# Autodesk Inventor assembly: camMounted
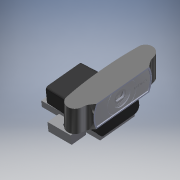
[picture p0: Inventor's stored thumbnail of the model, 180x180]
Saved by Autodesk Inventor 2017 (Build 210142000, 142)
## iProperties
Created: 2017-03-20
Part Number: camMounted
Document SubType Name: Assembly
Designer: Naga
Author: Naga
## Documents named in this file (3)
- E:\GDrive\IEEE CS\SoutheastCon2017\Cad\Electronics\camera\camMounted.iam
- E:\GDrive\IEEE CS\SoutheastCon2017\Cad\Electronics\camera\mount.ipt
- E:\GDrive\IEEE CS\SoutheastCon2017\Cad\Electronics\camera\LogitechC920Montaj.ipt
## Components (2 placed, 2 different names)
1. mount:1 — Mate:1, Mate:2, Flush:1
2. LogitechC920Montaj:1 — Mate:1, Mate:2, Flush:1
## Relationships (3: Mate 2, Flush 1)
- Mate:1: mount:1 ↔ LogitechC920Montaj:1
- Mate:2: mount:1 ↔ LogitechC920Montaj:1
- Flush:1 (-2.9083 mm): mount:1 ↔ LogitechC920Montaj:1
